# Autodesk Inventor assembly: Assembly
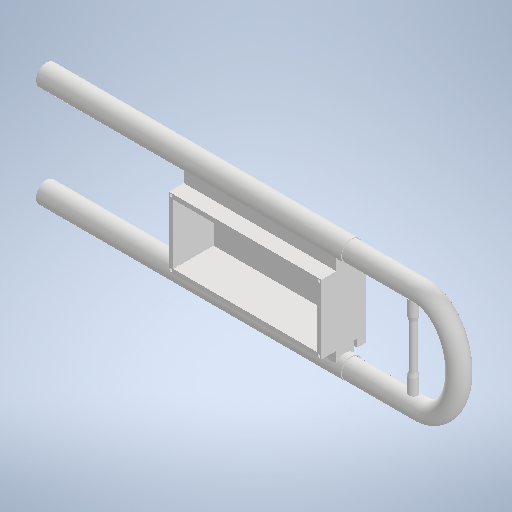
[picture p0: Inventor's stored thumbnail of the model, 512x512]
Saved by Autodesk Inventor 2025 (Build 290162010, 162A)
## iProperties
Created: 2025-01-21
Part Number: Assembly
Document SubType Name: Assembly
Designer: armenanzasn25
Author: armenanzasn25
## Documents named in this file (4)
- D:\Assembly.iam
- D:\Trumpet.ipt
- D:\Slide.ipt
- D:\Casing.ipt
## Components (3 placed, 3 different names)
1. Trumpet:1 — Cylindrical:1, Cylindrical:2
2. Slide:1 — Cylindrical:1
3. Casing:1 — Cylindrical:2
## Relationships (2: CylindricalJoint 2)
- Cylindrical:1: Trumpet:1 ↔ Slide:1
- Cylindrical:2: Trumpet:1 ↔ Casing:1
